# Autodesk Inventor assembly: HbSizeM
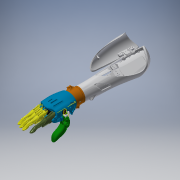
[picture p0: Inventor's stored thumbnail of the model, 180x180]
Saved by Autodesk Inventor 2018.2 (Build 222227000, 227)
## iProperties
Created: 2018-03-09
Part Number: HbSizeM
Material: 一般
Document SubType Name: Assembly
Designer: sktom
Author: sktom
## Documents named in this file (4)
- D:\CloudStrage\OneDrive\CADMech\HbSizeMMech\HbSizeM.iam
- D:\CloudStrage\OneDrive\CADMech\HbSizeMMech\UnitHand\Unit_MR-H\Unit_MR-H.iam
- D:\CloudStrage\OneDrive\CADMech\HbSizeMMech\UnitWrist\Unit_MR-W.iam
- D:\CloudStrage\OneDrive\CADMech\HbSizeMMech\UnitSocket\Unit_MR-SO.iam
## Components (3 placed, 3 different names)
1. Unit_MR-H:1 [sub-assembly] — 挿入:3
2. Unit_MR-W:1 [sub-assembly] — 挿入:1, 挿入:2, 挿入:3
3. Unit_MR-SO:1 [sub-assembly] — 挿入:1, 挿入:2
## Relationships (3: Insert 3)
- 挿入:1 [Insert]: Unit_MR-W:1 ↔ Unit_MR-SO:1
- 挿入:2 [Insert]: Unit_MR-W:1 ↔ Unit_MR-SO:1
- 挿入:3 [Insert]: Unit_MR-H:1 ↔ Unit_MR-W:1
